# Autodesk Inventor assembly: Assembly4
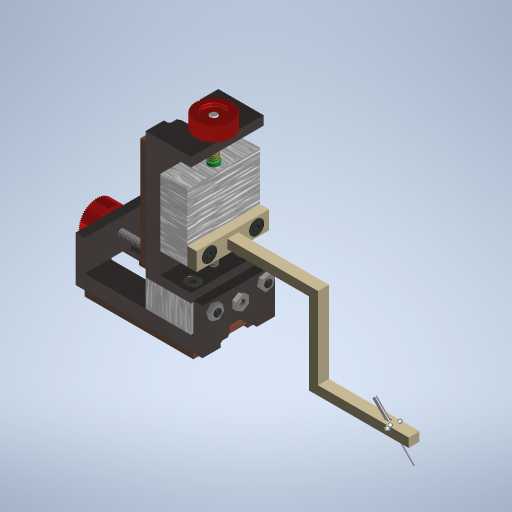
[picture p0: Inventor's stored thumbnail of the model, 512x512]
Saved by Autodesk Inventor 2024.3 (Build 283343010, 343A)
## iProperties
Part Number: Assembly4
Document SubType Name: Assembly
Designer: ACER
Author: ACER
## Documents named in this file (18)
- C:\Users\ACER\Desktop\project_copy_template_2024\Dhruv_1005859\1_Konstruktion\Assembly4.iam
- C:\Users\ACER\Desktop\project_copy_template_2024\Dhruv_1005859\1_Konstruktion\Base 3.ipt
- C:\Users\ACER\Desktop\project_copy_template_2024\Dhruv_1005859\1_Konstruktion\X_Slider_3.ipt
- C:\Users\ACER\Desktop\project_copy_template_2024\Dhruv_1005859\1_Konstruktion\Rail_Plate.ipt
- C:\Users\ACER\Desktop\project_copy_template_2024\Dhruv_1005859\1_Konstruktion\Z_Slider 3.ipt
- C:\Users\ACER\Desktop\project_copy_template_2024\Dhruv_1005859\1_Konstruktion\Lead Screw.ipt
- C:\Users\ACER\Desktop\project_copy_template_2024\Dhruv_1005859\1_Konstruktion\Knob.ipt
- C:\Users\ACER\Desktop\project_copy_template_2024\Dhruv_1005859\1_Konstruktion\Collar.ipt
- C:\Users\ACER\Desktop\project_copy_template_2024\Dhruv_1005859\1_Konstruktion\Rail_Holder 1.ipt
- C:\Users\ACER\Desktop\project_copy_template_2024\Dhruv_1005859\1_Konstruktion\Anti backlash Part 1.ipt
- C:\Users\ACER\Desktop\project_copy_template_2024\Dhruv_1005859\1_Konstruktion\Anti Backlash Part 2.ipt
- C:\Users\ACER\Desktop\project_copy_template_2024\Dhruv_1005859\1_Konstruktion\Spring.ipt
- C:\Users\ACER\Desktop\project_copy_template_2024\Dhruv_1005859\2_Normteile\en-US\ISO 10642(1)\ISO 10642 - M4 x  10.ipt
- C:\Users\ACER\Desktop\project_copy_template_2024\Dhruv_1005859\2_Normteile\en-US\AS 1474(1)\AS 1474 - M4(1).ipt
- C:\Users\ACER\Desktop\project_copy_template_2024\Dhruv_1005859\1_Konstruktion\Probe Arm.ipt
- C:\Users\ACER\Desktop\project_copy_template_2024\Dhruv_1005859\1_Konstruktion\ProbeTip.ipt
- C:\Users\ACER\Desktop\project_copy_template_2024\Dhruv_1005859\2_Normteile\en-US\DIN 913\DIN 913 - M1.4 x 2.5.ipt
- C:\Users\ACER\Desktop\project_copy_template_2024\Dhruv_1005859\2_Normteile\en-US\ISO 10642(1)\ISO 10642 - M4 x  8.ipt
## Components (48 placed, 17 different names)
1. Base 3:1 — Mate:1, Mate:3, Mate:48, Mate:60, Mate:69, Mate:70, Mate:71, Mate:72, Mate:73, Mate:74, Cylindrical:1, Cylindrical:2, Cylindrical:4, Cylindrical:5, Mate:87, Rotational:5, Mate:92, Mate:93, Mate:108, Mate:109, Cylindrical:17, Cylindrical:18, Rotational:7, Rotational:8
2. X_Slider_3:2 — Mate:1, Mate:3, Mate:5, Mate:6, Mate:7, Mate:33, Mate:34, Mate:37, Mate:41, Mate:46, Rotation/Translation:1, Rotational:6, Cylindrical:12, Mate:104, Mate:105, Cylindrical:15, Cylindrical:16
3. Base 3:2 — Mate:5, Mate:6, Mate:7, Mate:8, Mate:9, Mate:57, Mate:64, Mate:65, Mate:66, Mate:67, Mate:68, Cylindrical:8, Cylindrical:9, Cylindrical:10, Cylindrical:11, Mate:86, Rotational:4, Mate:91
4. Z_Slider 3:1 — Mate:8, Mate:9, Mate:35, Mate:36, Mate:39, Mate:40, Mate:58, Cylindrical:6, Cylindrical:7, Rotation/Translation:2, Rigid:3, Mate:94, Mate:95
5. Rail_Holder 1:2 — Mate:60, Mate:104, Mate:105, Mate:106, Mate:107
6. Rail_Plate:1 — Mate:64, Mate:65, Mate:84, Mate:85
7. Rail_Plate:2 — Mate:66, Mate:67, Mate:68, Mate:82, Mate:83
8. Rail_Plate:3 — Mate:71, Mate:72, Mate:73, Mate:80, Mate:81
9. Rail_Plate:4 — Mate:69, Mate:70, Mate:74, Mate:78, Mate:98
10. Knob:1 — Rigid:1
11. Knob:2 — Rigid:2
12. Lead Screw:1 — Mate:51, Mate:54, Mate:86, Rotational:4, Rigid:2, Rotation/Translation:2
13. Lead Screw:2 — Rigid:1, Mate:87, Rotational:5, Mate:88, Rotation/Translation:1
14. Collar:1 — Mate:35, Mate:36
15. Collar:2 — Mate:33, Mate:34
16. Collar:3 — Mate:39, Mate:40
17. Collar:4 — Mate:37, Mate:41
18. Anti backlash Part 1:1 — Mate:42, Mate:43, Mate:44, Mate:47, Mate:48, Mate:88
19. Anti Backlash Part 2:1 — Mate:43, Mate:44, Mate:46
20. Spring:1 — Mate:42, Mate:47
21. Anti backlash Part 1:2 — Mate:49, Mate:50, Mate:57
22. Anti Backlash Part 2:2 — Mate:49, Mate:50, Mate:51, Mate:55, Mate:56, Mate:58
23. Spring:2 — Mate:54, Mate:55, Mate:56
24. ISO 10642 M4x10:1 — Cylindrical:15, Mate:106
25. ISO 10642 M4x10:2 — Cylindrical:2, Mate:78
26. ISO 10642 M4x10:3 — Cylindrical:4, Mate:81
27. ISO 10642 M4x10:4 — Cylindrical:7, Mate:90
28. ISO 10642 M4x10:5 — Cylindrical:1, Mate:98
29. ISO 10642 M4x10:6 — Cylindrical:16, Mate:107
30. ISO 10642 M4x10:7 — Cylindrical:6, Mate:89
31. ISO 10642 M4x10:8 — Cylindrical:5, Mate:80
32. ISO 10642 M4x10:9 — Cylindrical:10, Mate:82
33. ISO 10642 M4x10:10 — Cylindrical:11, Mate:83
34. ISO 10642 M4x10:11 — Cylindrical:9, Mate:85
35. ISO 10642 M4x10:12 — Cylindrical:8, Mate:84
36. Rail_Holder 1:3 — Rigid:3, Mate:89, Mate:90
37. ISO 10642 M4x10:13 — Cylindrical:12, Mate:91
38. ISO 10642 M4x10:14 — Rotational:6
39. AS 1474 - Metric M4:1 — Mate:92, Mate:93
40. Probe Arm:1 — Mate:94, Mate:95, Cylindrical:13, Mate:96, Cylindrical:14, Mate:97, Mate:99, Mate:100, Mate:101, Mate:102, Mate:103
41. ISO 10642 M4x10:15 — Cylindrical:14, Mate:97
42. ISO 10642 M4x10:16 — Cylindrical:13, Mate:96
43. ProbeTip:1 — Mate:99, Mate:100, Mate:101
44. DIN 913 M1.4 x 2.5:1 — Mate:102, Mate:103
45. ISO 10642 M4x8:1 — Mate:108, Cylindrical:17
46. ISO 10642 M4x8:2 — Mate:109, Cylindrical:18
47. AS 1474 - Metric M4:2 — Rotational:7
48. AS 1474 - Metric M4:3 — Rotational:8
## Relationships (99: Mate 72, CylindricalJoint 17, RevoluteJoint 5, WeldJoint 3, RelateRotateTranslate 2)
- Mate:1: Base 3:1 ↔ X_Slider_3:2
- Mate:3: Base 3:1 ↔ X_Slider_3:2
- Mate:5: X_Slider_3:2 ↔ Base 3:2
- Mate:6: X_Slider_3:2 ↔ Base 3:2
- Mate:7: X_Slider_3:2 ↔ Base 3:2
- Mate:8: Base 3:2 ↔ Z_Slider 3:1
- Mate:9: Base 3:2 ↔ Z_Slider 3:1
- Rigid:1 [WeldJoint]: Knob:1 ↔ Lead Screw:2
- Mate:33: X_Slider_3:2 ↔ Collar:2
- Mate:34 (0.1 mm): X_Slider_3:2 ↔ Collar:2
- Mate:35: Z_Slider 3:1 ↔ Collar:1
- Mate:36 (0.1 mm): Z_Slider 3:1 ↔ Collar:1
- Mate:37: X_Slider_3:2 ↔ Collar:4
- Mate:39: Z_Slider 3:1 ↔ Collar:3
- Mate:40 (0.1 mm): Z_Slider 3:1 ↔ Collar:3
- Mate:41 (0.1 mm): X_Slider_3:2 ↔ Collar:4
- Mate:42: Anti backlash Part 1:1 ↔ Spring:1
- Mate:43 (1.5 mm): Anti backlash Part 1:1 ↔ Anti Backlash Part 2:1
- Mate:44: Anti backlash Part 1:1 ↔ Anti Backlash Part 2:1
- Mate:46: X_Slider_3:2 ↔ Anti Backlash Part 2:1
- Mate:47: Anti backlash Part 1:1 ↔ Spring:1
- Mate:48: Base 3:1 ↔ Anti backlash Part 1:1
- Mate:49: Anti backlash Part 1:2 ↔ Anti Backlash Part 2:2
- Mate:50 (1.5 mm): Anti backlash Part 1:2 ↔ Anti Backlash Part 2:2
- Mate:51: Lead Screw:1 ↔ Anti Backlash Part 2:2
- Mate:54: Lead Screw:1 ↔ Spring:2
- Mate:55: Anti Backlash Part 2:2 ↔ Spring:2
- Mate:56: Anti Backlash Part 2:2 ↔ Spring:2
- Mate:57: Base 3:2 ↔ Anti backlash Part 1:2
- Mate:58: Z_Slider 3:1 ↔ Anti Backlash Part 2:2
- Mate:60: Base 3:1 ↔ Rail_Holder 1:2
- Mate:64: Base 3:2 ↔ Rail_Plate:1
- Mate:65: Base 3:2 ↔ Rail_Plate:1
- Mate:66: Base 3:2 ↔ Rail_Plate:2
- Mate:67: Base 3:2 ↔ Rail_Plate:2
- Mate:68: Base 3:2 ↔ Rail_Plate:2
- Mate:69: Base 3:1 ↔ Rail_Plate:4
- Mate:70: Base 3:1 ↔ Rail_Plate:4
- Mate:71: Base 3:1 ↔ Rail_Plate:3
- Mate:72: Base 3:1 ↔ Rail_Plate:3
- Mate:73: Base 3:1 ↔ Rail_Plate:3
- Mate:74: Base 3:1 ↔ Rail_Plate:4
- Cylindrical:1: Base 3:1 ↔ ISO 10642 M4x10:5
- Cylindrical:2: Base 3:1 ↔ ISO 10642 M4x10:2
- Cylindrical:4: Base 3:1 ↔ ISO 10642 M4x10:3
- Cylindrical:5: Base 3:1 ↔ ISO 10642 M4x10:8
- Cylindrical:6: Z_Slider 3:1 ↔ ISO 10642 M4x10:7
- Cylindrical:7: Z_Slider 3:1 ↔ ISO 10642 M4x10:4
- Mate:78: Rail_Plate:4 ↔ ISO 10642 M4x10:2
- Mate:80: Rail_Plate:3 ↔ ISO 10642 M4x10:8
- Mate:81: Rail_Plate:3 ↔ ISO 10642 M4x10:3
- Cylindrical:8: Base 3:2 ↔ ISO 10642 M4x10:12
- Cylindrical:9: Base 3:2 ↔ ISO 10642 M4x10:11
- Cylindrical:10: Base 3:2 ↔ ISO 10642 M4x10:9
- Cylindrical:11: Base 3:2 ↔ ISO 10642 M4x10:10
- Mate:82: Rail_Plate:2 ↔ ISO 10642 M4x10:9
- Mate:83: Rail_Plate:2 ↔ ISO 10642 M4x10:10
- Mate:84: Rail_Plate:1 ↔ ISO 10642 M4x10:12
- Mate:85: Rail_Plate:1 ↔ ISO 10642 M4x10:11
- Mate:86: Base 3:2 ↔ Lead Screw:1
- Rotational:4 [RevoluteJoint]: Base 3:2 ↔ Lead Screw:1
- Rigid:2 [WeldJoint]: Knob:2 ↔ Lead Screw:1
- Mate:87: Base 3:1 ↔ Lead Screw:2
- Rotational:5 [RevoluteJoint]: Base 3:1 ↔ Lead Screw:2
- Mate:88: Lead Screw:2 ↔ Anti backlash Part 1:1
- Rotation/Translation:1 [RelateRotateTranslate] (24 mm): X_Slider_3:2 ↔ Lead Screw:2
- Rotation/Translation:2 [RelateRotateTranslate] (12 mm): Z_Slider 3:1 ↔ Lead Screw:1
- Rigid:3 [WeldJoint]: Z_Slider 3:1 ↔ Rail_Holder 1:3
- Mate:89: ISO 10642 M4x10:7 ↔ Rail_Holder 1:3
- Mate:90: ISO 10642 M4x10:4 ↔ Rail_Holder 1:3
- Rotational:6 [RevoluteJoint]: X_Slider_3:2 ↔ ISO 10642 M4x10:14
- Cylindrical:12: X_Slider_3:2 ↔ ISO 10642 M4x10:13
- Mate:91: Base 3:2 ↔ ISO 10642 M4x10:13
- Mate:92: Base 3:1 ↔ AS 1474 - Metric M4:1
- Mate:93: Base 3:1 ↔ AS 1474 - Metric M4:1
- Mate:94: Z_Slider 3:1 ↔ Probe Arm:1
- Mate:95: Z_Slider 3:1 ↔ Probe Arm:1
- Cylindrical:13: Probe Arm:1 ↔ ISO 10642 M4x10:16
- Mate:96: Probe Arm:1 ↔ ISO 10642 M4x10:16
- Cylindrical:14: Probe Arm:1 ↔ ISO 10642 M4x10:15
- Mate:97: Probe Arm:1 ↔ ISO 10642 M4x10:15
- Mate:98: Rail_Plate:4 ↔ ISO 10642 M4x10:5
- Mate:99 (1 mm): Probe Arm:1 ↔ ProbeTip:1
- Mate:100 (1 mm): Probe Arm:1 ↔ ProbeTip:1
- Mate:101: Probe Arm:1 ↔ ProbeTip:1
- Mate:102: Probe Arm:1 ↔ DIN 913 M1.4 x 2.5:1
- Mate:103: Probe Arm:1 ↔ DIN 913 M1.4 x 2.5:1
- Mate:104: X_Slider_3:2 ↔ Rail_Holder 1:2
- Mate:105: X_Slider_3:2 ↔ Rail_Holder 1:2
- Cylindrical:15: X_Slider_3:2 ↔ ISO 10642 M4x10:1
- Cylindrical:16: X_Slider_3:2 ↔ ISO 10642 M4x10:6
- Mate:106: Rail_Holder 1:2 ↔ ISO 10642 M4x10:1
- Mate:107: Rail_Holder 1:2 ↔ ISO 10642 M4x10:6
- Mate:108: Base 3:1 ↔ ISO 10642 M4x8:1
- Mate:109: Base 3:1 ↔ ISO 10642 M4x8:2
- Cylindrical:17: Base 3:1 ↔ ISO 10642 M4x8:1
- Cylindrical:18: Base 3:1 ↔ ISO 10642 M4x8:2
- Rotational:7 [RevoluteJoint]: Base 3:1 ↔ AS 1474 - Metric M4:2
- Rotational:8 [RevoluteJoint]: Base 3:1 ↔ AS 1474 - Metric M4:3
